# Autodesk Inventor assembly: 3030bracket
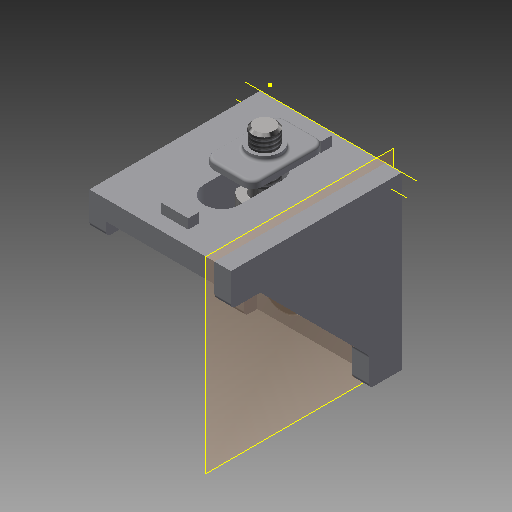
[picture p0: Inventor's stored thumbnail of the model, 512x512]
Saved by Autodesk Inventor 2017 (Build 210142000, 142)
## iProperties
Created: 2016-07-21
Part Number: 3030bracket
Document SubType Name: Assembly
Designer: User
Author: User
## Documents named in this file (5)
- C:\All INVENTOR\SL-Inventor\SL-Beast 3D Printer\3030bracket.iam
- C:\All INVENTOR\SL-Inventor\SL-Beast 3D Printer\30mm Bracket_CPY.ipt
- C:\All INVENTOR\SL-Inventor\SL-Beast 3D Printer\en-US\ANSI B18.3.1M(6)\ANSI B18.3.1M - M5x0.8 x 12(1).ipt
- C:\All INVENTOR\SL-Inventor\SL-Beast 3D Printer\en-US\ANSI B18.3.1M(6)\ANSI B18.3.1M - M6x1 x 10(1).ipt
- C:\All INVENTOR\SL-Inventor\SL-Beast 3D Printer\M5 Tee Nut_MIR_MIR.ipt
## Components (5 placed, 4 different names)
1. 30mm Bracket_CPY:1
2. Forged Socket Head Cap Screw - Metric M5x0.8 x 12:1
3. Forged Socket Head Cap Screw - Metric M6x1 x 10:1
4. M5 Tee Nut_MIR_MIR:1
5. M5 Tee Nut_MIR_MIR:2
## Relationships (5: Mate 4, Insert 1)
- [Mate]: 30mm Bracket_CPY:1 ↔ Forged Socket Head Cap Screw - Metric M5x0.8 x 12:1
- [Mate]: 30mm Bracket_CPY:1 ↔ Forged Socket Head Cap Screw - Metric M5x0.8 x 12:1
- [Insert]: 30mm Bracket_CPY:1 ↔ Forged Socket Head Cap Screw - Metric M6x1 x 10:1
- [Mate]: Forged Socket Head Cap Screw - Metric M5x0.8 x 12:1 ↔ M5 Tee Nut_MIR_MIR:1
- [Mate]: Forged Socket Head Cap Screw - Metric M6x1 x 10:1 ↔ M5 Tee Nut_MIR_MIR:2
